# Autodesk Inventor assembly: 足全体
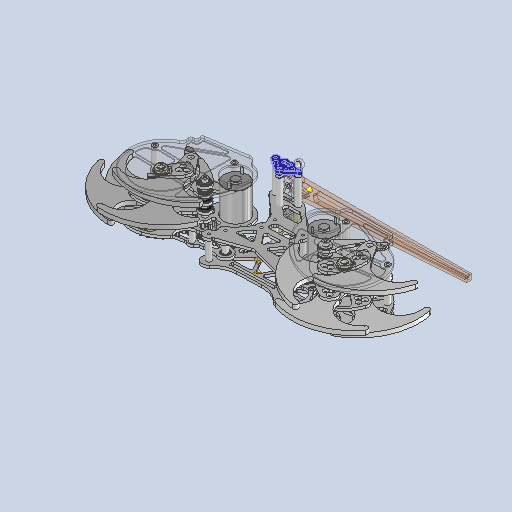
[picture p0: Inventor's stored thumbnail of the model, 512x512]
Saved by Autodesk Inventor 2023 (Build 270158000, 158)
## iProperties
Created: 2022-01-30
Part Number: 足全体
Document SubType Name: Assembly
Designer: acps
Mass: 767.98 g
Surface Area: 2765.24 cm^2
Volume: 318.532 cm^3
Density: 2.411 g/cm^3
Author: acps
## Documents named in this file (19)
- C:\Users\muzho\Documents\srdc\srdc_2\脚\足全体.iam
- C:\Users\muzho\Documents\srdc\srdc_2\脚\足ユニット.iam
- C:\Users\muzho\Documents\srdc\srdc_2\スペーサ\l23.ipt
- C:\Users\muzho\Documents\srdc\srdc_2\タミヤダンパー1.iam
- C:\Users\muzho\Documents\srdc\srdc_2\スペーサ\l10.ipt
- C:\Users\muzho\Documents\srdc\srdc_2\脚\中間ユニット内_MIR1.ipt
- C:\Users\muzho\Documents\srdc\srdc_2\スペーサ\l7.ipt
- C:\Users\muzho\Documents\srdc\srdc_2\脚\足ユニット_MIR.iam
- C:\Users\muzho\Documents\srdc\srdc_2\脚\ミラー\l10_MIR.ipt
- C:\Users\muzho\Documents\srdc\srdc_2\脚\ミラー\l7_MIR.ipt
- C:\Users\muzho\Documents\srdc\srdc_2\スペーサ\l3.ipt
- C:\Users\muzho\Documents\srdc\srdc_2\スペーサ\l23_peak.ipt
- C:\Users\muzho\Documents\srdc\srdc_2\スペーサ\l30.ipt
- C:\Users\muzho\Documents\srdc\srdc_2\脚\ウィング関連\足 横wing下板 .ipt
- C:\Users\muzho\Documents\srdc\srdc_2\脚\ウィング関連\足 横wing固定用外フレーム.ipt
- C:\Users\muzho\Documents\srdc\srdc_2\脚\中間ユニット外(shin)_MIR.ipt
- C:\Users\muzho\Documents\srdc\srdc_2\スペーサ\l12.ipt
- C:\Users\muzho\Documents\srdc\srdc_2\脚\ウィング関連\横wing 押さえ.ipt
- C:\Users\muzho\Documents\srdc\srdc_2\脚\ウィング関連\横wing _MIR.ipt
## Components (33 placed, 18 different names)
1. 足ユニット:1 [sub-assembly] — 挿入:17, 挿入:23
2. l23:1 — 挿入:33
3. l23:2 — 挿入:32
4. l23:3 — 挿入:35
5. l23:4 — 挿入:16
6. l23:5 — 挿入:28
7. l23:6 — 挿入:19
8. l23:7 — 挿入:22
9. l23:8 — 挿入:20
10. タミヤダンパー1:1 [sub-assembly] — 挿入:24
11. l10:1 — 挿入:23, 挿入:24
12. 中間ユニット内_MIR1:1 — 挿入:16, 挿入:17, 挿入:19, 挿入:20, 挿入:22, 挿入:25, 挿入:28, 挿入:31, 挿入:32, 挿入:33, 挿入:35, フラッシュ:1, メイト:9, メイト:10, 挿入:36, 挿入:37, 挿入:38
13. l7:1 — 挿入:25
14. 足ユニット_MIR:1 [sub-assembly] — 挿入:34
15. l10_MIR:1 — メイト:8, 挿入:30, 挿入:34
16. l7_MIR:1 — 挿入:31
17. タミヤダンパー1:2 [sub-assembly] — メイト:8, 挿入:30
18. l3:1 — 挿入:43
19. l3:2 — 挿入:42, 挿入:45
20. l3:3 — 挿入:44, メイト:11, 挿入:48
21. l23_peak:1 — 挿入:38
22. l23_peak:2 — 挿入:37, メイト:13
23. l23_peak:3 — 挿入:36, メイト:12, 挿入:46
24. l30:1 — 挿入:44
25. l30:2 — 挿入:42, 挿入:47
26. l30:3 — 挿入:43
27. 足 横wing下板 :1 — フラッシュ:1, メイト:9, メイト:10, 挿入:49, 挿入:50, メイト:17
28. 足 横wing固定用外フレーム:1 — メイト:11, 挿入:45, 挿入:48
29. 中間ユニット外(shin)_MIR:1 — メイト:12, メイト:13, 挿入:46, 挿入:47
30. l12:1 — 挿入:50, 挿入:51, メイト:16
31. l12:2 — 挿入:49, メイト:14, メイト:15
32. 横wing 押さえ:1 — メイト:14, 挿入:51
33. 横wing _MIR:1 — メイト:15, メイト:16, メイト:17
## Relationships (39: Insert 28, Mate 10, Flush 1)
- 挿入:16 [Insert]: l23:4 ↔ 中間ユニット内_MIR1:1
- 挿入:17 [Insert]: 足ユニット:1 ↔ 中間ユニット内_MIR1:1
- 挿入:19 [Insert]: l23:6 ↔ 中間ユニット内_MIR1:1
- 挿入:20 [Insert]: l23:8 ↔ 中間ユニット内_MIR1:1
- 挿入:22 [Insert]: l23:7 ↔ 中間ユニット内_MIR1:1
- 挿入:23 [Insert]: 足ユニット:1 ↔ l10:1
- 挿入:24 [Insert]: タミヤダンパー1:1 ↔ l10:1
- 挿入:25 [Insert]: 中間ユニット内_MIR1:1 ↔ l7:1
- 挿入:28 [Insert]: l23:5 ↔ 中間ユニット内_MIR1:1
- メイト:8 [Mate]: l10_MIR:1 ↔ タミヤダンパー1:2
- 挿入:30 [Insert]: l10_MIR:1 ↔ タミヤダンパー1:2
- 挿入:31 [Insert]: 中間ユニット内_MIR1:1 ↔ l7_MIR:1
- 挿入:32 [Insert]: l23:2 ↔ 中間ユニット内_MIR1:1
- 挿入:33 [Insert]: l23:1 ↔ 中間ユニット内_MIR1:1
- 挿入:34 [Insert]: 足ユニット_MIR:1 ↔ l10_MIR:1
- 挿入:35 [Insert]: l23:3 ↔ 中間ユニット内_MIR1:1
- フラッシュ:1 [Flush]: 中間ユニット内_MIR1:1 ↔ 足 横wing下板 :1
- メイト:9 [Mate]: 中間ユニット内_MIR1:1 ↔ 足 横wing下板 :1
- メイト:10 [Mate]: 中間ユニット内_MIR1:1 ↔ 足 横wing下板 :1
- 挿入:36 [Insert]: 中間ユニット内_MIR1:1 ↔ l23_peak:3
- 挿入:37 [Insert]: 中間ユニット内_MIR1:1 ↔ l23_peak:2
- 挿入:38 [Insert]: 中間ユニット内_MIR1:1 ↔ l23_peak:1
- 挿入:42 [Insert]: l3:2 ↔ l30:2
- 挿入:43 [Insert]: l3:1 ↔ l30:3
- 挿入:44 [Insert]: l3:3 ↔ l30:1
- メイト:11 [Mate]: l3:3 ↔ 足 横wing固定用外フレーム:1
- 挿入:45 [Insert]: l3:2 ↔ 足 横wing固定用外フレーム:1
- メイト:12 [Mate]: l23_peak:3 ↔ 中間ユニット外(shin)_MIR:1
- メイト:13 [Mate]: l23_peak:2 ↔ 中間ユニット外(shin)_MIR:1
- 挿入:46 [Insert]: l23_peak:3 ↔ 中間ユニット外(shin)_MIR:1
- 挿入:47 [Insert]: l30:2 ↔ 中間ユニット外(shin)_MIR:1
- 挿入:48 [Insert]: l3:3 ↔ 足 横wing固定用外フレーム:1
- 挿入:49 [Insert]: 足 横wing下板 :1 ↔ l12:2
- 挿入:50 [Insert]: 足 横wing下板 :1 ↔ l12:1
- メイト:14 [Mate]: l12:2 ↔ 横wing 押さえ:1
- 挿入:51 [Insert]: l12:1 ↔ 横wing 押さえ:1
- メイト:15 [Mate]: l12:2 ↔ 横wing _MIR:1
- メイト:16 [Mate]: l12:1 ↔ 横wing _MIR:1
- メイト:17 [Mate] (5 mm): 足 横wing下板 :1 ↔ 横wing _MIR:1
